# Autodesk Inventor assembly: 20-J2
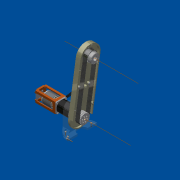
[picture p0: Inventor's stored thumbnail of the model, 180x180]
Saved by Autodesk Inventor 2018 (Build 220112000, 112)
## iProperties
Created: 2020-01-14
Part Number: 20-J2
Document SubType Name: Assembly
Designer: Bunny320
Author: Bunny320
## Documents named in this file (10)
- D:\Seerosenstr\sechs\4-CAD\30-J3.iam
- D:\Seerosenstr\sechs\4-CAD\201-flange-with motor.ipt
- D:\Seerosenstr\sechs\4-CAD\standardParts\61807-2RS1\61807-2RS1.iam
- D:\Seerosenstr\sechs\4-CAD\motor unit.iam
- D:\Seerosenstr\sechs\4-CAD\generated\J3_belt.iam
- C:\Users\mo\Documents\Inventor\Content Center Files\R2018\en-US\ISO 4762(1)\DIN EN ISO 4762 - M3 x 12.ipt
- C:\Users\mo\Documents\Inventor\Content Center Files\R2018\en-US\ISO 4762(1)\DIN EN ISO 4762 - M3 x 20.ipt
- D:\Seerosenstr\sechs\4-CAD\standardParts\Pololu mounting hub\pololu-universal-aluminum-mounting-hub-for-8mm-shaft-m3-holes.ipt
- D:\Seerosenstr\sechs\4-CAD\303-link right.ipt
- D:\Seerosenstr\sechs\4-CAD\standardParts\W 619_4-2Z\W 619_4-2Z.iam
## Components (14 placed, 9 different names)
1. 201-flange-with motor:1 — Flush:1, Flush:2, Flush:3, Mate:3, Mate:4, Mate:7, Mate:8, Mate:9, Mate:34, Mate:35, Mate:36, Mate:37, Mate:38, Mate:39, Mate:40, Mate:41, Mate:42, Mate:43
2. 61807-2RS1:1 [sub-assembly] — Mate:3, Mate:4, Mate:66, Mate:67
3. 61807-2RS1:2 [sub-assembly] — Mate:58, Mate:59, Mate:60
4. motor unit:1 [sub-assembly] — Mate:7, Mate:8, Mate:9, Mate:14, Mate:56
5. J3_belt:1 [sub-assembly] — Mate:14, Mate:57, Mate:60
6. DIN EN ISO 4762 M3 x 12:5 — Mate:34, Mate:35
7. DIN EN ISO 4762 M3 x 12:6 — Mate:36, Mate:37
8. DIN EN ISO 4762 M3 x 12:7 — Mate:38, Mate:39
9. DIN EN ISO 4762 M3 x 12:8 — Mate:40, Mate:41
10. DIN EN ISO 4762 M3 x 20:1 — Mate:42, Mate:43
11. pololu-universal-aluminum-mounting-hub-for-8mm-shaft-m3-holes:1 — Mate:56, Mate:57
12. 303-link right:1 — Mate:58, Mate:59, Mate:62, Mate:63, Mate:64, Mate:65, Mate:66, Mate:67
13. W 619_4-2Z:1 [sub-assembly] — Mate:62, Mate:64
14. W 619_4-2Z:2 [sub-assembly] — Mate:63, Mate:65
## Relationships (30: Mate 27, Flush 3)
- Flush:1: 201-flange-with motor:1
- Flush:2: 201-flange-with motor:1
- Flush:3: 201-flange-with motor:1
- Mate:3: 201-flange-with motor:1 ↔ 61807-2RS1:1
- Mate:4: 201-flange-with motor:1 ↔ 61807-2RS1:1
- Mate:7: 201-flange-with motor:1 ↔ motor unit:1
- Mate:8: 201-flange-with motor:1 ↔ motor unit:1
- Mate:9: 201-flange-with motor:1 ↔ motor unit:1
- Mate:14: motor unit:1 ↔ J3_belt:1
- Mate:34: 201-flange-with motor:1 ↔ DIN EN ISO 4762 M3 x 12:5
- Mate:35: 201-flange-with motor:1 ↔ DIN EN ISO 4762 M3 x 12:5
- Mate:36: 201-flange-with motor:1 ↔ DIN EN ISO 4762 M3 x 12:6
- Mate:37: 201-flange-with motor:1 ↔ DIN EN ISO 4762 M3 x 12:6
- Mate:38: 201-flange-with motor:1 ↔ DIN EN ISO 4762 M3 x 12:7
- Mate:39: 201-flange-with motor:1 ↔ DIN EN ISO 4762 M3 x 12:7
- Mate:40: 201-flange-with motor:1 ↔ DIN EN ISO 4762 M3 x 12:8
- Mate:41: 201-flange-with motor:1 ↔ DIN EN ISO 4762 M3 x 12:8
- Mate:42: 201-flange-with motor:1 ↔ DIN EN ISO 4762 M3 x 20:1
- Mate:43: 201-flange-with motor:1 ↔ DIN EN ISO 4762 M3 x 20:1
- Mate:56: motor unit:1 ↔ pololu-universal-aluminum-mounting-hub-for-8mm-shaft-m3-holes:1
- Mate:57: J3_belt:1 ↔ pololu-universal-aluminum-mounting-hub-for-8mm-shaft-m3-holes:1
- Mate:58: 61807-2RS1:2 ↔ 303-link right:1
- Mate:59: 61807-2RS1:2 ↔ 303-link right:1
- Mate:60: 61807-2RS1:2 ↔ J3_belt:1
- Mate:62: 303-link right:1 ↔ W 619_4-2Z:1
- Mate:63: 303-link right:1 ↔ W 619_4-2Z:2
- Mate:64: 303-link right:1 ↔ W 619_4-2Z:1
- Mate:65: 303-link right:1 ↔ W 619_4-2Z:2
- Mate:66: 61807-2RS1:1 ↔ 303-link right:1
- Mate:67: 61807-2RS1:1 ↔ 303-link right:1
